# Autodesk Inventor assembly: s-assy-pulley
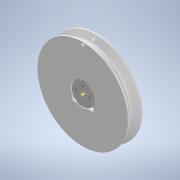
[picture p0: Inventor's stored thumbnail of the model, 180x180]
Saved by Autodesk Inventor 2022 (Build 260153000, 153)
## iProperties
Created: 2021-09-15
Part Number: s-assy-pulley
Document SubType Name: Assembly
Designer: yuto6
Author: yuto6
## Documents named in this file (3)
- C:\Users\yuto6\Box\Public_Share\キャチロボバトルコンテスト2021\CAD\catchrobo_hardware\assy-shooter\s-assy-shooter_pulley.iam
- C:\Users\yuto6\Box\Public_Share\キャチロボバトルコンテスト2021\CAD\catchrobo_hardware\assy-shooter\s_base7.ipt
- C:\Users\yuto6\Box\Public_Share\キャチロボバトルコンテスト2021\CAD\catchrobo_hardware\assy-shooter\SCSTR6-8.iam
## Components (2 placed, 2 different names)
1. s_base7:1 — メイト:1, メイト:2, メイト:3
2. SCSTR6-8:1 [sub-assembly] — メイト:1, メイト:2, メイト:3
## Relationships (3: Mate 3)
- メイト:1 [Mate]: s_base7:1 ↔ SCSTR6-8:1
- メイト:2 [Mate]: s_base7:1 ↔ SCSTR6-8:1
- メイト:3 [Mate]: s_base7:1 ↔ SCSTR6-8:1
